# Autodesk Inventor assembly: Assembly
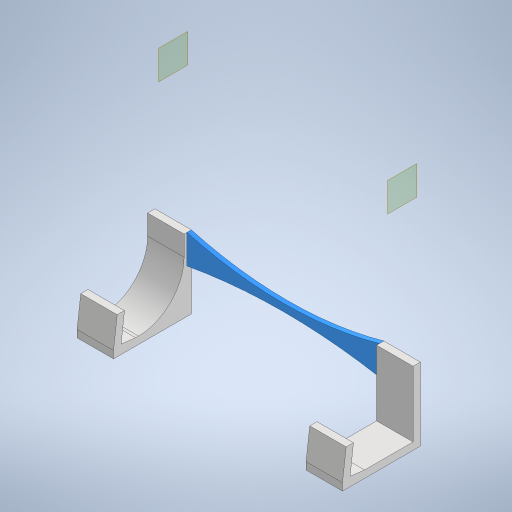
[picture p0: Inventor's stored thumbnail of the model, 512x512]
Saved by Autodesk Inventor 2023 (Build 270158000, 158)
## iProperties
Created: 2023-02-02
Part Number: Assembly
Document SubType Name: Assembly
Designer: shrey
Author: shrey
## Documents named in this file (6)
- D:\Inventor Projects\Wall Vinyl Cover Holder\Assembly.iam
- D:\Inventor Projects\Wall Vinyl Cover Holder\wall.ipt
- D:\Inventor Projects\Wall Vinyl Cover Holder\Album.ipt
- D:\Inventor Projects\Wall Vinyl Cover Holder\coverHolder.ipt
- D:\Inventor Projects\Wall Vinyl Cover Holder\spacer.ipt
- D:\Inventor Projects\Wall Vinyl Cover Holder\coverHolder_CPY.ipt
## Components (5 placed, 5 different names)
1. wall:1 — Flush:1, Mate:1, Mate:2, Angle:1, Mate:3
2. Album:1 — Flush:2, Angle:1, Mate:3, Angle:2
3. coverHolder:1 — Mate:4, Mate:5, Flush:3
4. spacer:1 — Mate:6, Mate:7, Flush:4
5. coverHolder(right):1 — Mate:8
## Relationships (14: Mate 8, Flush 4, Angle 2)
- Flush:1: wall:1
- Mate:1: wall:1
- Mate:2: wall:1
- Flush:2: Album:1
- Angle:1 (-7 deg): wall:1 ↔ Album:1
- Mate:3: wall:1 ↔ Album:1
- Angle:2 (-7 deg): Album:1
- Mate:4: coverHolder:1
- Mate:5: coverHolder:1
- Flush:3: coverHolder:1
- Mate:6: spacer:1
- Mate:7: spacer:1
- Flush:4: spacer:1
- Mate:8 (157.15 mm): coverHolder(right):1
